# Autodesk Inventor assembly: Intake 2.0 MASTER
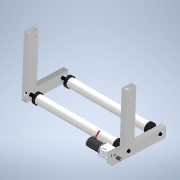
[picture p0: Inventor's stored thumbnail of the model, 180x180]
Saved by Autodesk Inventor 2020 (Build 240168000, 168)
## iProperties
Created: 2020-01-26
Part Number: Intake 2.0 MASTER
Document SubType Name: Assembly
Designer: autum
Author: autum
## Documents named in this file (6)
- \\CSSDFS03\Student_k$\1cikaychapman\My Documents\Downloads\Robot 2020\Intake 2.0\Intake 2.0 MASTER.iam
- \\CSSDFS03\Student_k$\1cikaychapman\My Documents\Downloads\Robot 2020\Intake 2.0\Roller.iam
- \\CSSDFS03\Student_k$\1cikaychapman\My Documents\Downloads\Robot 2020\Intake 2.0\2x1 Top.ipt
- \\CSSDFS03\Student_k$\1cikaychapman\My Documents\Downloads\Robot 2020\Intake 2.0\2x1 Front.ipt
- \\CSSDFS03\Student_k$\1cikaychapman\My Documents\Downloads\Robot 2020\Intake 2.0\2x1 Front with motor mount.ipt
- \\CSSDFS03\Student_k$\1cikaychapman\My Documents\Downloads\Robot 2020\Intake 2.0\VersaPlanetary_v2_Single_Stage_10_1_with_BAG.iam
## Components (7 placed, 5 different names)
1. Roller:1 [sub-assembly] — Insert:1
2. Roller:2 [sub-assembly] — Insert:2
3. 2x1 Top:1 — Flush:5, Flush:6, Mate:3, Mate:6, Flush:7
4. 2x1 Top:2 — Mate:1, Flush:1, Flush:2, Flush:5, Flush:6, Mate:3
5. 2x1 Front:2 — Mate:1, Flush:1, Flush:2, Flush:8
6. 2x1 Front with motor mount:1 — Mate:6, Flush:7, Flush:8, Insert:1, Insert:2, Mate:7, Flush:9, Flush:10
7. VersaPlanetary_v2_Single_Stage_10_1_with_BAG:1 [sub-assembly] — Mate:7, Flush:9, Flush:10
## Relationships (14: Flush 8, Mate 4, Insert 2)
- Mate:1: 2x1 Top:2 ↔ 2x1 Front:2
- Flush:1: 2x1 Top:2 ↔ 2x1 Front:2
- Flush:2: 2x1 Top:2 ↔ 2x1 Front:2
- Flush:5: 2x1 Top:1 ↔ 2x1 Top:2
- Flush:6: 2x1 Top:1 ↔ 2x1 Top:2
- Mate:3 (482.6 mm): 2x1 Top:1 ↔ 2x1 Top:2
- Mate:6: 2x1 Top:1 ↔ 2x1 Front with motor mount:1
- Flush:7: 2x1 Top:1 ↔ 2x1 Front with motor mount:1
- Flush:8: 2x1 Front:2 ↔ 2x1 Front with motor mount:1
- Insert:1 (25.4 mm): Roller:1 ↔ 2x1 Front with motor mount:1
- Insert:2 (25.4 mm): Roller:2 ↔ 2x1 Front with motor mount:1
- Mate:7: 2x1 Front with motor mount:1 ↔ VersaPlanetary_v2_Single_Stage_10_1_with_BAG:1
- Flush:9 (5.08 mm): 2x1 Front with motor mount:1 ↔ VersaPlanetary_v2_Single_Stage_10_1_with_BAG:1
- Flush:10 (3.81 mm): 2x1 Front with motor mount:1 ↔ VersaPlanetary_v2_Single_Stage_10_1_with_BAG:1
